# Autodesk Inventor assembly: SERVO
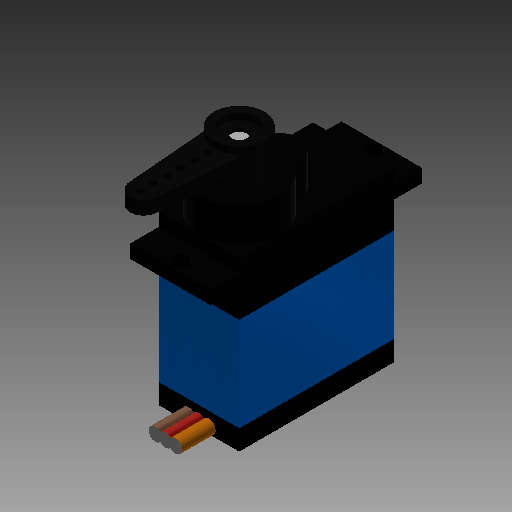
[picture p0: Inventor's stored thumbnail of the model, 512x512]
Saved by Autodesk Inventor 2017.3 (Build 213256000, 256)
## iProperties
Created: 2017-09-24
Part Number: SERVO
Document SubType Name: Assembly
Designer: Alexander Miller
Author: Alexander Miller
## Documents named in this file (3)
- X:\Alex\Documents\Git\HeRo-Mini\Hardware\SERVO.iam
- X:\Alex\Documents\Git\HeRo-Mini\Hardware\TP-MG92B.ipt
- X:\Alex\Documents\Git\HeRo-Mini\Hardware\TP-MG92B_HAT.ipt
## Components (2 placed, 2 different names)
1. TP-MG92B:1 — Rotational:1
2. TP-MG92B_HAT:1 — Rotational:1
## Relationships (1: RevoluteJoint 1)
- Rotational:1 [RevoluteJoint]: TP-MG92B:1 ↔ TP-MG92B_HAT:1
